# Autodesk Inventor assembly: Фильтр D1200
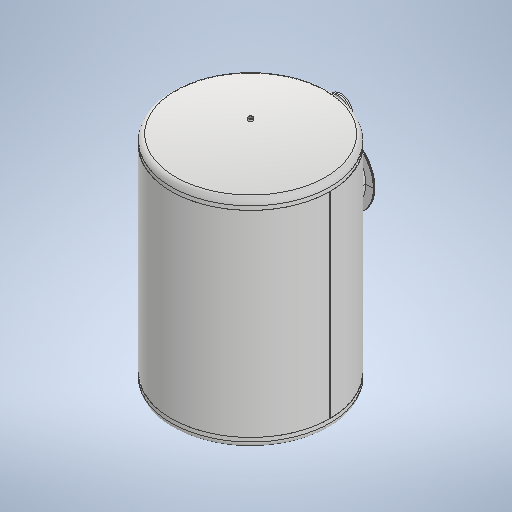
[picture p0: Inventor's stored thumbnail of the model, 512x512]
Saved by Autodesk Inventor 2025 (Build 290162010, 162A)
## iProperties
Created: 2025-02-13
Part Number: Фильтр D1200
Document SubType Name: Assembly
Designer: pokla
Author: pokla
## Documents named in this file (11)
- C:\Users\pokla\Desktop\Работа Акватроник\Фильтры напорные\D1200\ASY Фильтр D1200.iam
- C:\Users\pokla\Desktop\Работа Акватроник\Фильтры напорные\D1200\Заглушка ревиз. окна фильтра D1200.ipt
- C:\Users\pokla\Desktop\Работа Акватроник\Фильтры напорные\D1200\Заглушка фланца трубы подключения фильтра D1200.ipt
- C:\Users\pokla\Desktop\Работа Акватроник\Фильтры напорные\D1200\Кольцо заглушки ревиз. окна фильтра D1200.ipt
- C:\Users\pokla\Desktop\Работа Акватроник\Фильтры напорные\D1200\Размеры D1200.ipt
- C:\Users\pokla\Desktop\Работа Акватроник\Фильтры напорные\D1200\Ревиз. окно фильтра D1200.ipt
- C:\Users\pokla\Desktop\Работа Акватроник\Фильтры напорные\D1200\Стенка фильтра D1200.ipt
- C:\Users\pokla\Desktop\Работа Акватроник\Фильтры напорные\D1200\Труба подключения фильтра D1200.ipt
- C:\Users\pokla\Desktop\Работа Акватроник\Фильтры напорные\D1200\Фланец трубы подключения фильтра D1200.ipt
- C:\Users\pokla\Desktop\Работа Акватроник\Фильтры напорные\D1200\Сферическое дно D1200.ipt
- C:\Users\pokla\Desktop\Работа Акватроник\Фильтры напорные\D1200\Штуцер фильтра D1200.ipt
## Components (18 placed, 10 different names)
1. Заглушка ревиз. окна фильтра D1200:1 — Rigid:12
2. Заглушка фланца трубы подключения фильтра D1200:1 — Rigid:19
3. Кольцо заглушки ревиз. окна фильтра D1200:1 — Rigid:1, Rigid:11
4. Размеры D1200:1
5. Ревиз. окно фильтра D1200:1 — Rigid:10, Rigid:11, Rigid:12
6. Стенка фильтра D1200:1 — Rigid:5, Rigid:9, Rigid:10, Rigid:13, Rigid:14
7. Труба подключения фильтра D1200:1 — Rigid:3, Rigid:5, Rigid:17, Rigid:19
8. Фланец трубы подключения фильтра D1200:1 — Rigid:17
9. Кольцо заглушки ревиз. окна фильтра D1200:2 — Rigid:1
10. Фланец трубы подключения фильтра D1200:2 — Rigid:3
11. Заглушка фланца трубы подключения фильтра D1200:2 — Rigid:20
12. Труба подключения фильтра D1200:2 — Rigid:9, Rigid:18, Rigid:20
13. Фланец трубы подключения фильтра D1200:3 — Rigid:18
14. Фланец трубы подключения фильтра D1200:4
15. Сферическое дно D1200:1 — Rigid:13, Rigid:16
16. Сферическое дно D1200:2 — Rigid:14, Rigid:15
17. Штуцер фильтра D1200:1 — Rigid:15
18. Штуцер фильтра D1200:2 — Rigid:16
## Relationships (16: WeldJoint 16)
- Rigid:1 [WeldJoint]: Кольцо заглушки ревиз. окна фильтра D1200:1 ↔ Кольцо заглушки ревиз. окна фильтра D1200:2
- Rigid:3 [WeldJoint]: Труба подключения фильтра D1200:1 ↔ Фланец трубы подключения фильтра D1200:2
- Rigid:5 [WeldJoint] (97 mm): Стенка фильтра D1200:1 ↔ Труба подключения фильтра D1200:1
- [WeldJoint]: Труба подключения фильтра D1200:2 ↔ Фланец трубы подключения фильтра D1200:4
- Rigid:9 [WeldJoint] (97 mm): Стенка фильтра D1200:1 ↔ Труба подключения фильтра D1200:2
- Rigid:10 [WeldJoint] (66 mm): Ревиз. окно фильтра D1200:1 ↔ Стенка фильтра D1200:1
- Rigid:11 [WeldJoint]: Кольцо заглушки ревиз. окна фильтра D1200:1 ↔ Ревиз. окно фильтра D1200:1
- Rigid:12 [WeldJoint]: Заглушка ревиз. окна фильтра D1200:1 ↔ Ревиз. окно фильтра D1200:1
- Rigid:13 [WeldJoint]: Стенка фильтра D1200:1 ↔ Сферическое дно D1200:1
- Rigid:14 [WeldJoint]: Стенка фильтра D1200:1 ↔ Сферическое дно D1200:2
- Rigid:15 [WeldJoint]: Сферическое дно D1200:2 ↔ Штуцер фильтра D1200:1
- Rigid:16 [WeldJoint]: Сферическое дно D1200:1 ↔ Штуцер фильтра D1200:2
- Rigid:17 [WeldJoint]: Труба подключения фильтра D1200:1 ↔ Фланец трубы подключения фильтра D1200:1
- Rigid:18 [WeldJoint]: Труба подключения фильтра D1200:2 ↔ Фланец трубы подключения фильтра D1200:3
- Rigid:19 [WeldJoint]: Заглушка фланца трубы подключения фильтра D1200:1 ↔ Труба подключения фильтра D1200:1
- Rigid:20 [WeldJoint]: Заглушка фланца трубы подключения фильтра D1200:2 ↔ Труба подключения фильтра D1200:2
## Named parameters: d7_d2 = 0 mm
